# Autodesk Inventor assembly: Ensamblaje3
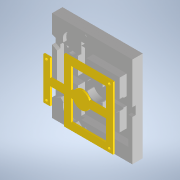
[picture p0: Inventor's stored thumbnail of the model, 180x180]
Saved by Autodesk Inventor 2021 (Build 250183000, 183)
## iProperties
Created: 2022-11-05
Part Number: Ensamblaje3
Document SubType Name: Assembly
Designer: ivanm
Author: ivanm
## Documents named in this file (5)
- C:\Users\ivanm\OneDrive\Servomecanismos\Proyectos\Proyecto academico\Servomecanismo2R\INVENTOR\Ensamblaje3.iam
- C:\Users\ivanm\OneDrive\Servomecanismos\Proyectos\Proyecto academico\Servomecanismo2R\INVENTOR\TablaBase.ipt
- C:\Users\ivanm\OneDrive\Servomecanismos\Proyectos\Proyecto academico\Servomecanismo2R\INVENTOR\Etapa2Base.ipt
- C:\Users\ivanm\OneDrive\Servomecanismos\Proyectos\Proyecto academico\Servomecanismo2R\INVENTOR\ParteFinalMesaEnsamble.ipt
- C:\Users\ivanm\OneDrive\Robotica\Proyecto-Rob\Piezas\BaseGripper.ipt
## Components (4 placed, 4 different names)
1. TablaBase:1 — Nivelación:1, Nivelación:2, Coincidencia:1
2. Etapa2Base:1 — Nivelación:1, Nivelación:2, Coincidencia:1, Coincidencia:2, Nivelación:3, Nivelación:4
3. ParteFinalMesaEnsamble:1 — Coincidencia:2, Nivelación:3, Nivelación:4
4. BaseGripper:1
## Relationships (6: Flush 4, Mate 2)
- Nivelación:1 [Flush]: TablaBase:1 ↔ Etapa2Base:1
- Nivelación:2 [Flush]: TablaBase:1 ↔ Etapa2Base:1
- Coincidencia:1 [Mate]: TablaBase:1 ↔ Etapa2Base:1
- Coincidencia:2 [Mate]: Etapa2Base:1 ↔ ParteFinalMesaEnsamble:1
- Nivelación:3 [Flush]: Etapa2Base:1 ↔ ParteFinalMesaEnsamble:1
- Nivelación:4 [Flush]: Etapa2Base:1 ↔ ParteFinalMesaEnsamble:1
